# Autodesk Inventor assembly: Tracking Assy
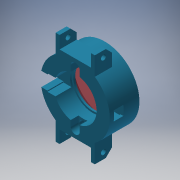
[picture p0: Inventor's stored thumbnail of the model, 180x180]
Saved by Autodesk Inventor 2016 (Build 200138000, 138)
## iProperties
Created: 2016-04-05
Part Number: Tracking Assy
Document SubType Name: Assembly
Designer: xdlea
Author: xdlea
## Documents named in this file (3)
- C:\Users\xdlea\Documents\3D Models\Tracking Assy.iam
- C:\Users\xdlea\Documents\3D Models\Glass.ipt
- C:\Users\xdlea\Documents\3D Models\Tracking Bracelet.ipt
## Components (2 placed, 2 different names)
1. Glass:1 — Mate:1, Mate:2
2. Tracking Bracelet:1 — Mate:1, Mate:2
## Relationships (2: Mate 2)
- Mate:1: Glass:1 ↔ Tracking Bracelet:1
- Mate:2: Glass:1 ↔ Tracking Bracelet:1
